# Autodesk Inventor assembly: Assembly2
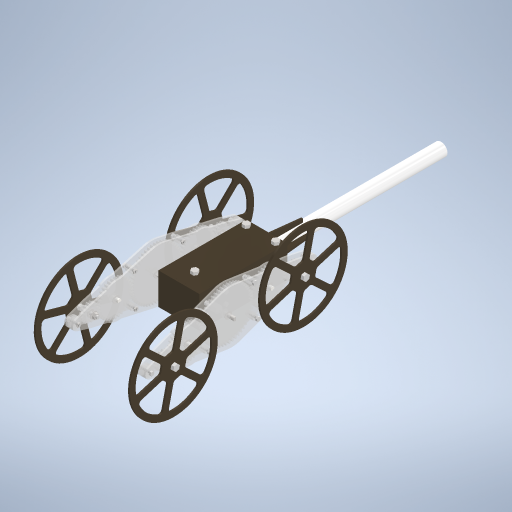
[picture p0: Inventor's stored thumbnail of the model, 512x512]
Saved by Autodesk Inventor 2023 (Build 270158000, 158)
## iProperties
Created: 2023-07-30
Part Number: Assembly2
Document SubType Name: Assembly
Designer: Ronan
Author: Ronan
## Documents named in this file (2)
- D:\Libraries\Documents\2023-FYP\Inventor\Assembly v2\Assembly2.iam
- D:\Libraries\Documents\2023-FYP\Inventor\Assembly v2\Assembly.iam
## Components (1 placed, 1 different names)
1. Assembly:1 [sub-assembly] — Flush:1, Flush:2
## Relationships (2: Flush 2)
- Flush:1: Assembly:1
- Flush:2: Assembly:1
